# Autodesk Inventor assembly: s-assy-idler3
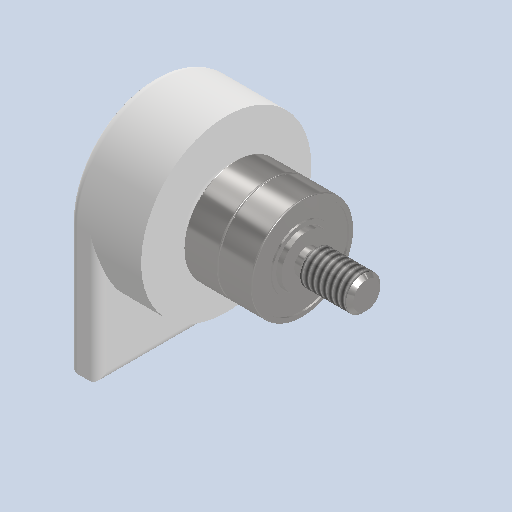
[picture p0: Inventor's stored thumbnail of the model, 512x512]
Saved by Autodesk Inventor 2022 (Build 260153000, 153)
## iProperties
Created: 2022-06-14
Part Number: s-assy-idler3
Document SubType Name: Assembly
Designer: yuto6
Author: yuto6
## Documents named in this file (4)
- C:\Users\yuto6\Documents\CAD\book-reader\s-assy-idler3.iam
- C:\Users\yuto6\Documents\CAD\book-reader\MR126ZZ.ipt
- C:\Users\yuto6\Documents\CAD\book-reader\MSB6-15.ipt
- C:\Users\yuto6\Documents\CAD\book-reader\base8.ipt
## Components (4 placed, 3 different names)
1. MR126ZZ:1 — メイト:3, メイト:4, メイト:8
2. MR126ZZ:2 — メイト:3, メイト:5
3. MSB6-15:1 — メイト:4, メイト:5, メイト:6, メイト:7
4. base8:1 — メイト:6, メイト:7, メイト:8
## Relationships (6: Mate 6)
- メイト:3 [Mate]: MR126ZZ:1 ↔ MR126ZZ:2
- メイト:4 [Mate]: MR126ZZ:1 ↔ MSB6-15:1
- メイト:5 [Mate]: MR126ZZ:2 ↔ MSB6-15:1
- メイト:6 [Mate]: MSB6-15:1 ↔ base8:1
- メイト:7 [Mate]: MSB6-15:1 ↔ base8:1
- メイト:8 [Mate]: MR126ZZ:1 ↔ base8:1
